# Autodesk Inventor assembly: Left Angle Structure
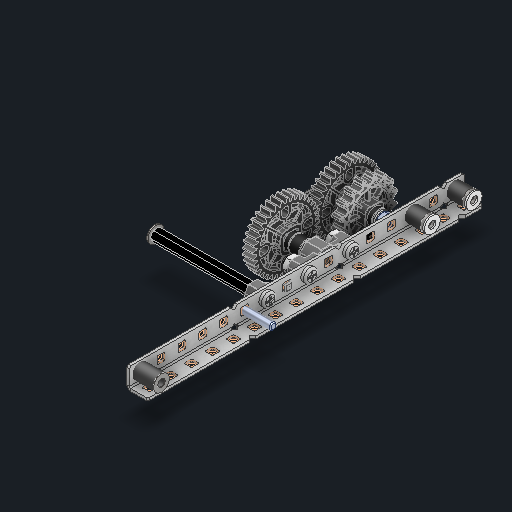
[picture p0: Inventor's stored thumbnail of the model, 512x512]
Saved by Autodesk Inventor 2025.1 (Build 291241000, 241)
## iProperties
Created: 2024-10-20
Part Number: Left Angle Structure
Document SubType Name: Assembly
Designer: Averey Ku
Author: Averey Ku
## Documents named in this file (23)
- C:\Users\avere\VEX\High Stakes\CAD\V3\Intake\Left Angle Structure.iam
- C:\Users\avere\VEX\High Stakes\CAD\ROBOPROS-CAD-Inventor\Motion\Spacers\Spacer Nylon .375 OD\NSpacer .375 OD x .375.ipt
- C:\Users\avere\VEX\High Stakes\CAD\ROBOPROS-CAD-Inventor\Motion\Spacers\Washer Steel\SWasher .375 OD x .062500.ipt
- C:\Users\avere\VEX\High Stakes\CAD\ROBOPROS-CAD-Inventor\Motion\Spacers\Washer Teflon\TWasher .375 OD x .04000.ipt
- C:\Users\avere\VEX\High Stakes\CAD\ROBOPROS-CAD-Inventor\Structure\Angle\Aluminum 1x1\Alu Angle 1x1x16.ipt
- C:\Users\avere\VEX\High Stakes\CAD\ROBOPROS-CAD-Inventor\Motion\Spacers\Spacer Nylon .375 OD\NSpacer .375 OD x .500.ipt
- C:\Users\avere\VEX\High Stakes\CAD\ROBOPROS-CAD-Inventor\Motion\Spacers\Washer Steel\SWasher .375 OD x .015625.ipt
- C:\Users\avere\VEX\High Stakes\CAD\ROBOPROS-CAD-Inventor\Motion\Shaft HS\HS Bearing Flat.ipt
- C:\Users\avere\VEX\High Stakes\CAD\ROBOPROS-CAD-Inventor\Structure\Hardware\Nut Nylon\Nut Nylon - White.ipt
- C:\Users\avere\VEX\High Stakes\CAD\V3\Intake\Gearbox.iam
- Gearbox Left.iam
- C:\Users\avere\VEX\High Stakes\CAD\ROBOPROS-CAD-Inventor\Motion\Spacers\Spacer Nylon .375 OD.ipt
- C:\Users\avere\VEX\High Stakes\CAD\ROBOPROS-CAD-Inventor\Motion\Spacers\Washer Steel.ipt
- C:\Users\avere\VEX\High Stakes\CAD\ROBOPROS-CAD-Inventor\Structure\Hardware\Nut Nylon.ipt
- C:\Users\avere\VEX\High Stakes\CAD\ROBOPROS-CAD-Inventor\Motion\Spacers\Washer Teflon.ipt
- C:\Users\avere\VEX\High Stakes\CAD\ROBOPROS-CAD-Inventor\Structure\1-Post Standoff Retainer.ipt
- C:\Users\avere\VEX\High Stakes\CAD\ROBOPROS-CAD-Inventor\Structure\Standoff\Standoff 2.50.ipt
- C:\Users\avere\VEX\High Stakes\CAD\ROBOPROS-CAD-Inventor\Structure\Standoff.ipt
- C:\Users\avere\VEX\High Stakes\CAD\ROBOPROS-CAD-Inventor\Structure\Hardware\Screw Nylon - Pan Head\NScrew Pan Head Threaded .375.ipt
- C:\Users\avere\VEX\High Stakes\CAD\ROBOPROS-CAD-Inventor\Motion\Spacers\Washer Steel\SWasher .375 OD x .031250.ipt
- C:\Users\avere\VEX\High Stakes\CAD\ROBOPROS-CAD-Inventor\Structure\Hardware\Screw Nylon - Pan Head\NScrew Pan Head Threaded .500.ipt
- C:\Users\avere\VEX\High Stakes\CAD\ROBOPROS-CAD-Inventor\Structure\Hardware\Screw Steel - Star\SScrew Star Smooth .750.ipt
- C:\Users\avere\VEX\High Stakes\CAD\ROBOPROS-CAD-Inventor\Structure\Hardware\Screw Steel - Star.ipt
## Components (20 placed, 15 different names)
1. Alu Angle 1x1x16:1 — Flush:1, Mate:1, Mate:2, Insert:3, Insert:4, Mate:4, Insert:11, Insert:14, Insert:17, Mate:5, Insert:20, Insert:21, Insert:23, Insert:24, Mate:7
2. NSpacer .375 OD x .500:1 — Insert:2, Insert:3
3. SWasher .375 OD x .015625:1 — Insert:2
4. HS Bearing Flat:1 — Insert:4, Mate:4, Insert:5, Insert:6
5. Nut Nylon - White:1 — Insert:5
6. Nut Nylon - White:2 — Insert:6
7. NSpacer .375 OD x .375:2 — Insert:10, Insert:11
8. SWasher .375 OD x .062500:2 — Insert:9, Insert:10
9. TWasher .375 OD x .04000:1 — Insert:9
10. NSpacer .375 OD x .375:3 — Insert:14
11. SWasher .375 OD x .062500:3
12. TWasher .375 OD x .04000:2
13. Gearbox Left:1 [sub-assembly] — Insert:24, Mate:7
14. 1-Post Standoff Retainer:1 — Insert:16, Angle:1, Insert:17, Mate:5, Insert:18
15. Standoff 2.50:1 — Insert:16, Angle:1, Insert:19
16. NScrew Pan Head Threaded .375:1 — Insert:18
17. SWasher .375 OD x .031250:4 — Insert:19
18. NScrew Pan Head Threaded .500:1 — Insert:21
19. NScrew Pan Head Threaded .500:2 — Insert:20
20. SScrew Star Smooth .750:1 — Insert:23
## Relationships (26: Insert 19, Mate 5, Flush 1, Angle 1)
- Flush:1 (-101.6 mm): Alu Angle 1x1x16:1
- Mate:1: Alu Angle 1x1x16:1
- Mate:2: Alu Angle 1x1x16:1
- Insert:2: NSpacer .375 OD x .500:1 ↔ SWasher .375 OD x .015625:1
- Insert:3: Alu Angle 1x1x16:1 ↔ NSpacer .375 OD x .500:1
- Insert:4: Alu Angle 1x1x16:1 ↔ HS Bearing Flat:1
- Mate:4: Alu Angle 1x1x16:1 ↔ HS Bearing Flat:1
- Insert:5: HS Bearing Flat:1 ↔ Nut Nylon - White:1
- Insert:6: HS Bearing Flat:1 ↔ Nut Nylon - White:2
- Insert:9: SWasher .375 OD x .062500:2 ↔ TWasher .375 OD x .04000:1
- Insert:10: NSpacer .375 OD x .375:2 ↔ SWasher .375 OD x .062500:2
- Insert:11: Alu Angle 1x1x16:1 ↔ NSpacer .375 OD x .375:2
- [Insert]: SWasher .375 OD x .062500:3 ↔ TWasher .375 OD x .04000:2
- [Insert]: NSpacer .375 OD x .375:3 ↔ SWasher .375 OD x .062500:3
- Insert:14: Alu Angle 1x1x16:1 ↔ NSpacer .375 OD x .375:3
- Insert:16: 1-Post Standoff Retainer:1 ↔ Standoff 2.50:1
- Angle:1 (0 deg): 1-Post Standoff Retainer:1 ↔ Standoff 2.50:1
- Insert:17: Alu Angle 1x1x16:1 ↔ 1-Post Standoff Retainer:1
- Mate:5: Alu Angle 1x1x16:1 ↔ 1-Post Standoff Retainer:1
- Insert:18 (1.5875 mm): 1-Post Standoff Retainer:1 ↔ NScrew Pan Head Threaded .375:1
- Insert:19: Standoff 2.50:1 ↔ SWasher .375 OD x .031250:4
- Insert:20: Alu Angle 1x1x16:1 ↔ NScrew Pan Head Threaded .500:2
- Insert:21: Alu Angle 1x1x16:1 ↔ NScrew Pan Head Threaded .500:1
- Insert:23: Alu Angle 1x1x16:1 ↔ SScrew Star Smooth .750:1
- Insert:24: Alu Angle 1x1x16:1 ↔ Gearbox Left:1
- Mate:7: Alu Angle 1x1x16:1 ↔ Gearbox Left:1
## Named parameters: d40_d37 = 0 mm, d41_d38 = 0 mm
